# Autodesk Inventor assembly: omni_platformav222
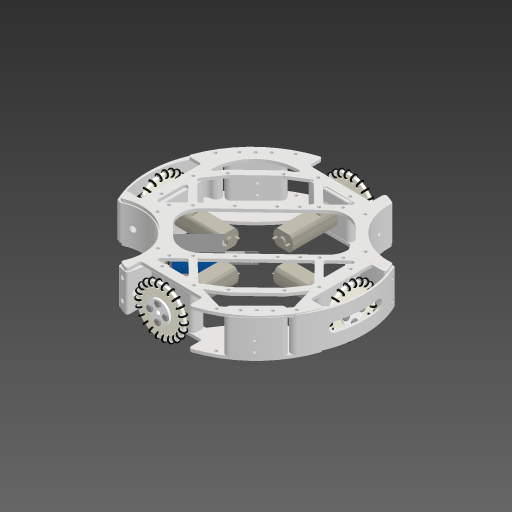
[picture p0: Inventor's stored thumbnail of the model, 512x512]
Saved by Autodesk Inventor 2023 (Build 270158000, 158)
## iProperties
Created: 2025-09-23
Part Number: omni_platformav222
Document SubType Name: Assembly
Designer: daa
Author: daa
## Documents named in this file (9)
- C:\Users\daa\Documents\DASH_V2\omni_platforma\omni_platformav222.iam
- C:\Users\daa\Documents\DASH_V2\omni_platforma\bottom.ipt
- C:\Users\daa\Documents\DASH_V2\omni_platforma\motor_sb.iam
- C:\Users\daa\Documents\DASH_V2\omni_platforma\handle mount.ipt
- C:\Users\daa\Documents\DASH_V2\omni_platforma\Solenoid.iam
- C:\Users\daa\Documents\DASH_V2\omni_platforma\ball_solenoid_v2.ipt
- C:\Users\daa\Documents\DASH_V2\omni_platforma\dribler_ball.ipt
- C:\Users\daa\Documents\DASH_V2\omni_platforma\protect_2.ipt
- C:\Users\daa\Documents\DASH_V2\omni_platforma\top_v2.ipt
## Components (13 placed, 8 different names)
1. bottom:1 — Совмещение:1, Совмещение:2, Совмещение:3, С поворотом:1, Совмещение:4, Совмещение:5, Совмещение:6, Совмещение:7, Совмещение:8, Совмещение:9, Совмещение:10, Совмещение:11, С поворотом:2, Совмещение:12, Совмещение:13, Совмещение:14, Совмещение:15, Совмещение:16, С поворотом:3
2. motor_sb:1 [sub-assembly] — Совмещение:3, С поворотом:1
3. motor_sb:2 [sub-assembly] — Совмещение:6, Совмещение:7
4. motor_sb:3 [sub-assembly] — Совмещение:4, Совмещение:5
5. motor_sb:4 [sub-assembly] — Совмещение:1, Совмещение:2
6. handle mount:1 — Совмещение:10, Совмещение:11
7. handle mount:2 — Совмещение:8, Совмещение:9
8. Solenoid:1 [sub-assembly] — С поворотом:2
9. ball_solenoid_v2:1 — Совмещение:12, Совмещение:13, Совмещение:17
10. dribler_ball:1 — Совмещение:14, Совмещение:15, Совмещение:18
11. protect_2:1 — Совмещение:16
12. protect_2:2 — С поворотом:3
13. top_v2:1 — Совмещение:17, Совмещение:18
## Relationships (21: Mate 18, RevoluteJoint 3)
- Совмещение:1 [Mate]: bottom:1 ↔ motor_sb:4
- Совмещение:2 [Mate]: bottom:1 ↔ motor_sb:4
- Совмещение:3 [Mate]: bottom:1 ↔ motor_sb:1
- С поворотом:1 [RevoluteJoint]: bottom:1 ↔ motor_sb:1
- Совмещение:4 [Mate]: bottom:1 ↔ motor_sb:3
- Совмещение:5 [Mate]: bottom:1 ↔ motor_sb:3
- Совмещение:6 [Mate]: bottom:1 ↔ motor_sb:2
- Совмещение:7 [Mate]: bottom:1 ↔ motor_sb:2
- Совмещение:8 [Mate]: bottom:1 ↔ handle mount:2
- Совмещение:9 [Mate]: bottom:1 ↔ handle mount:2
- Совмещение:10 [Mate]: bottom:1 ↔ handle mount:1
- Совмещение:11 [Mate]: bottom:1 ↔ handle mount:1
- С поворотом:2 [RevoluteJoint]: bottom:1 ↔ Solenoid:1
- Совмещение:12 [Mate]: bottom:1 ↔ ball_solenoid_v2:1
- Совмещение:13 [Mate]: bottom:1 ↔ ball_solenoid_v2:1
- Совмещение:14 [Mate]: bottom:1 ↔ dribler_ball:1
- Совмещение:15 [Mate]: bottom:1 ↔ dribler_ball:1
- Совмещение:16 [Mate]: bottom:1 ↔ protect_2:1
- С поворотом:3 [RevoluteJoint]: bottom:1 ↔ protect_2:2
- Совмещение:17 [Mate]: ball_solenoid_v2:1 ↔ top_v2:1
- Совмещение:18 [Mate]: dribler_ball:1 ↔ top_v2:1
